# Autodesk Inventor assembly: Wheel
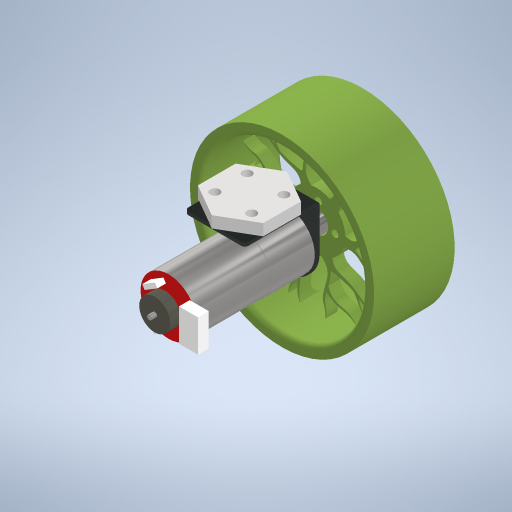
[picture p0: Inventor's stored thumbnail of the model, 512x512]
Saved by Autodesk Inventor 2024.2 (Build 282272000, 272)
## iProperties
Created: 2025-06-30
Part Number: Wheel
Document SubType Name: Assembly
Designer: Admin
Author: Admin
## Documents named in this file (6)
- C:\Users\Admin\Documents\GitHub\ExplorateurErrant\Assemblies\Wheel.iam
- C:\Users\Admin\Documents\GitHub\ExplorateurErrant\Motors\DC-JGA25\WH-Bracket-JGA25.ipt
- C:\Users\Admin\Documents\GitHub\ExplorateurErrant\Motors\DC-JGA25\WH-Motor-JGA25.ipt
- C:\Users\Admin\Documents\GitHub\ExplorateurErrant\Motors\DC-JGA25\WH-Coupling-4mm.ipt
- C:\Users\Admin\Documents\GitHub\ExplorateurErrant\Wheels\WH-SuspensionBounding-FirstApproach.ipt
- C:\Users\Admin\Documents\GitHub\ExplorateurErrant\Wheels\RhymTest.ipt
## Components (5 placed, 5 different names)
1. WH-Bracket-JGA25:1 — Mate:1, Mate:2, Mate:3, Mate:5, Mate:6, Mate:7
2. WH-Motor-JGA25:1 — Mate:1, Mate:2, Mate:3, Mate:4
3. WH-Coupling-4mm:1 — Mate:4, Mate:8, Mate:9, Mate:10
4. WH-SuspensionBounding-FirstApproach:1 — Mate:5, Mate:6, Mate:7
5. RhymTest:1 — Mate:8, Mate:9, Mate:10
## Relationships (10: Mate 10)
- Mate:1: WH-Bracket-JGA25:1 ↔ WH-Motor-JGA25:1
- Mate:2: WH-Bracket-JGA25:1 ↔ WH-Motor-JGA25:1
- Mate:3: WH-Bracket-JGA25:1 ↔ WH-Motor-JGA25:1
- Mate:4: WH-Motor-JGA25:1 ↔ WH-Coupling-4mm:1
- Mate:5: WH-Bracket-JGA25:1 ↔ WH-SuspensionBounding-FirstApproach:1
- Mate:6: WH-Bracket-JGA25:1 ↔ WH-SuspensionBounding-FirstApproach:1
- Mate:7: WH-Bracket-JGA25:1 ↔ WH-SuspensionBounding-FirstApproach:1
- Mate:8: WH-Coupling-4mm:1 ↔ RhymTest:1
- Mate:9: WH-Coupling-4mm:1 ↔ RhymTest:1
- Mate:10: WH-Coupling-4mm:1 ↔ RhymTest:1
